# Autodesk Inventor assembly: SprayCanAndServo
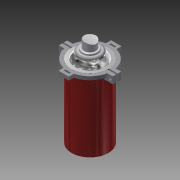
[picture p0: Inventor's stored thumbnail of the model, 180x180]
Saved by Autodesk Inventor 2014 SP1 (Build 180222100, 222)
## iProperties
Created: 2017-02-23
Part Number: SprayCanAndServo
Document SubType Name: Assembly
Designer: danielsikar
Author: danielsikar
## Documents named in this file (3)
- C:\Users\danielsikar\Documents\Projects\iot-graffiti\cad\assemblies\SprayCanAndServo.iam
- C:\Users\danielsikar\Documents\Projects\iot-graffiti\cad\parts\SprayCan105mm.ipt
- C:\Users\danielsikar\Documents\Projects\iot-graffiti\cad\parts\CanBracket.ipt
## Components (3 placed, 2 different names)
1. SprayCan105mm:1 — Flush:1, Flush:2, Flush:3, Mate:3, Mate:4, Mate:5
2. CanBracket:1 — Mate:1, Mate:2, Mate:3
3. CanBracket:2 — Mate:4, Flush:6, Mate:5
## Relationships (10: Flush 5, Mate 5)
- Flush:1: SprayCan105mm:1
- Flush:2: SprayCan105mm:1
- Flush:3: SprayCan105mm:1
- Mate:1 (100 mm): CanBracket:1
- Flush:4 (1 mm)
- Mate:2: CanBracket:1
- Mate:3: SprayCan105mm:1 ↔ CanBracket:1
- Mate:4 (100 mm): SprayCan105mm:1 ↔ CanBracket:2
- Flush:6 (2 mm): CanBracket:2
- Mate:5: SprayCan105mm:1 ↔ CanBracket:2
